# Autodesk Inventor assembly: fox
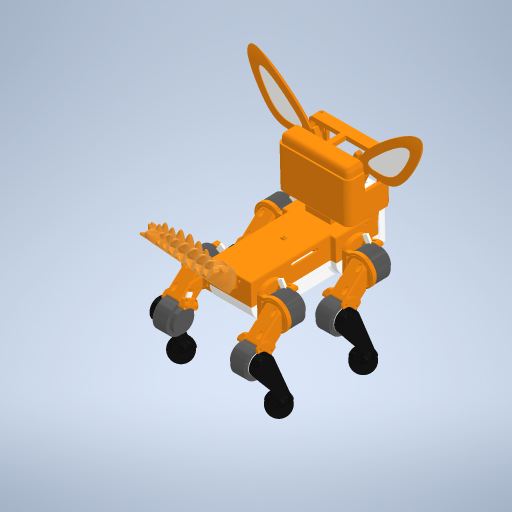
[picture p0: Inventor's stored thumbnail of the model, 512x512]
Saved by Autodesk Inventor 2024.2 (Build 282272000, 272)
## iProperties
Created: 2025-09-19
Part Number: fox
Document SubType Name: Assembly
Designer: AdminForWorker
Mass: 1852.12 g
Surface Area: 6976.59 cm^2
Volume: 1264.54 cm^3
Density: 1.46466 g/cm^3
d9: 11,000 мм
Title: Pupper v3.5 v16
Author: AdminForWorker
## Documents named in this file (16)
- D:\dog\fox\construction\fox\fox.iam
- D:\dog\fox\construction\fox\legs\Lower leg - Short Short V6 (No Pinch) v20.iam
- D:\dog\fox\construction\fox\legs\Lower leg - Short Short V6 (No Pinch) v20_1.iam
- D:\dog\fox\construction\fox\legs\две части ног.iam
- D:\dog\fox\construction\fox\body\тело лисы.iam
- D:\dog\fox\construction\fox\legs\одна часть ноги.iam
- D:\dog\fox\construction\fox\legs\одна часть ноги симетр.iam
- D:\dog\fox\construction\fox\legs\Lower leg - Short Short V6 (No Pinch) v20(Mirror).iam
- D:\dog\fox\construction\fox\legs\Lower leg - Short Short V6 (No Pinch) v20(Mirror)_1.iam
- D:\dog\fox\construction\fox\body\аккумулятор 21700.iam
- D:\dog\fox\construction\fox\body\хвост.ipt
- D:\dog\fox\construction\fox\body\аккумулятор 18650.iam
- D:\dog\fox\construction\fox\body\делать держит аккум.ipt
- D:\dog\fox\construction\fox\body\оси.ipt
- D:\dog\fox\docx\photos\кнопка.ipt
- D:\dog\fox\construction\fox\body\кнопка2часть.ipt
## Components (15 placed, 15 different names)
1. тело [sub-assembly] — Совмещение:1, Совмещение:2, Совмещение:4, Цилиндрический:1, Совмещение:5, Совмещение:6, Цилиндрический:2, С поворотом:1, С поворотом:2, Заподлицо:6, Совмещение:20, Заподлицо:13, Заподлицо:14, Совмещение:24
2. нижняя нога правая 2 [sub-assembly] — Совмещение:15, Совмещение:16
3. верхняя нога левая [sub-assembly] — Цилиндрический:1, Совмещение:5, Совмещение:6, Совмещение:15, Совмещение:16
4. верхняя нога правая [sub-assembly] — Совмещение:4, Цилиндрический:2, С поворотом:1, Совмещение:13, Совмещение:14
5. нижняя нога левая 2 [sub-assembly] — Совмещение:13, Совмещение:14
6. нижняя нога левая [sub-assembly] — С поворотом:3
7. нижняя нога правая [sub-assembly] — Совмещение:17, Совмещение:18
8. верхняя нога перед [sub-assembly] — С поворотом:2, С поворотом:3, Совмещение:17, Совмещение:18, Совмещение:24
9. аккумулятор 21700:1 [sub-assembly] — Совмещение:1, Совмещение:2
10. хвост:1
11. аккумулятор 18650:1 [sub-assembly] — Совмещение:20, Совмещение:21, Совмещение:23
12. делать держит аккум:1 — Совмещение:21, Совмещение:23
13. оси — Заподлицо:6
14. кнопка:1 — Заподлицо:13, Заподлицо:14, Заподлицо:15
15. кнопка2часть:1 — Заподлицо:15
## Relationships (24: Mate 15, Flush 4, RevoluteJoint 3, CylindricalJoint 2)
- Совмещение:1 [Mate] (4 mm): тело ↔ аккумулятор 21700:1
- Совмещение:2 [Mate] (11 mm): тело ↔ аккумулятор 21700:1
- Совмещение:4 [Mate]: тело ↔ верхняя нога правая
- Цилиндрический:1 [CylindricalJoint]: тело ↔ верхняя нога левая
- Совмещение:5 [Mate]: тело ↔ верхняя нога левая
- Совмещение:6 [Mate]: тело ↔ верхняя нога левая
- Цилиндрический:2 [CylindricalJoint]: тело ↔ верхняя нога правая
- С поворотом:1 [RevoluteJoint]: тело ↔ верхняя нога правая
- С поворотом:2 [RevoluteJoint]: тело ↔ верхняя нога перед
- С поворотом:3 [RevoluteJoint]: нижняя нога левая ↔ верхняя нога перед
- Совмещение:13 [Mate]: верхняя нога правая ↔ нижняя нога левая 2
- Совмещение:14 [Mate]: верхняя нога правая ↔ нижняя нога левая 2
- Совмещение:15 [Mate]: нижняя нога правая 2 ↔ верхняя нога левая
- Совмещение:16 [Mate]: нижняя нога правая 2 ↔ верхняя нога левая
- Совмещение:17 [Mate]: нижняя нога правая ↔ верхняя нога перед
- Совмещение:18 [Mate]: нижняя нога правая ↔ верхняя нога перед
- Заподлицо:6 [Flush]: тело ↔ оси
- Совмещение:20 [Mate]: тело ↔ аккумулятор 18650:1
- Совмещение:21 [Mate]: аккумулятор 18650:1 ↔ делать держит аккум:1
- Совмещение:23 [Mate]: аккумулятор 18650:1 ↔ делать держит аккум:1
- Заподлицо:13 [Flush]: тело ↔ кнопка:1
- Заподлицо:14 [Flush] (5 mm): тело ↔ кнопка:1
- Заподлицо:15 [Flush]: кнопка:1 ↔ кнопка2часть:1
- Совмещение:24 [Mate]: тело ↔ верхняя нога перед
